# Autodesk Inventor assembly: assembly-1
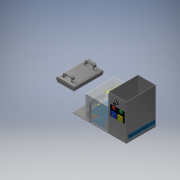
[picture p0: Inventor's stored thumbnail of the model, 180x180]
Saved by Autodesk Inventor 2019 (Build 230136000, 136)
## iProperties
Created: 2020-03-01
Part Number: assembly-1
Document SubType Name: Assembly
Designer: Hp
Author: Hp
## Documents named in this file (11)
- F:\2nd sem\INVENTOR\amit\amit 3d\assembly-1.iam
- F:\2nd sem\INVENTOR\amit\amit 3d\container.ipt
- F:\2nd sem\INVENTOR\amit\amit 3d\rack coloumn.ipt
- F:\2nd sem\INVENTOR\amit\amit 3d\Arduino MEGA 2560.ipt
- F:\2nd sem\INVENTOR\amit\amit 3d\PINION.ipt
- F:\2nd sem\INVENTOR\amit\amit 3d\dc motor.ipt
- F:\2nd sem\INVENTOR\amit\amit 3d\OUTER CASE.ipt
- F:\2nd sem\INVENTOR\amit\amit 3d\lid.ipt
- F:\2nd sem\INVENTOR\amit\amit 3d\IR SENSOR.ipt
- F:\2nd sem\INVENTOR\amit\amit 3d\BUZZER.ipt
- F:\2nd sem\INVENTOR\amit\amit 3d\conveyor 2.ipt
## Components (12 placed, 10 different names)
1. container:1 — Rigid:3, Rigid:5, Rigid:8, Rigid:12, Rigid:13, Rotational:2, Rigid:14
2. rack coloumn:1 — Rigid:3, Rigid:6
3. Arduino MEGA 2560:1 — Rigid:5
4. PINION:1 — Rigid:6, Rotational:1
5. dc motor:1 — Rotational:1
6. Arduino MEGA 2560:2 — Rigid:8
7. OUTER CASE:1
8. lid:1
9. IR SENSOR:1 — Rigid:12
10. IR SENSOR:2 — Rigid:13
11. BUZZER:1 — Rotational:2
12. conveyor 2:1 — Rigid:14
## Relationships (9: WeldJoint 7, RevoluteJoint 2)
- Rigid:3 [WeldJoint]: container:1 ↔ rack coloumn:1
- Rigid:5 [WeldJoint]: container:1 ↔ Arduino MEGA 2560:1
- Rigid:6 [WeldJoint]: rack coloumn:1 ↔ PINION:1
- Rotational:1 [RevoluteJoint]: PINION:1 ↔ dc motor:1
- Rigid:8 [WeldJoint]: container:1 ↔ Arduino MEGA 2560:2
- Rigid:12 [WeldJoint]: container:1 ↔ IR SENSOR:1
- Rigid:13 [WeldJoint]: container:1 ↔ IR SENSOR:2
- Rotational:2 [RevoluteJoint]: container:1 ↔ BUZZER:1
- Rigid:14 [WeldJoint]: container:1 ↔ conveyor 2:1
